# Autodesk Inventor assembly: martro_hettlich
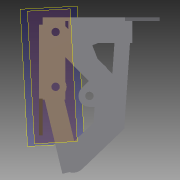
[picture p0: Inventor's stored thumbnail of the model, 180x180]
Saved by Autodesk Inventor 2015 SP1 (Build 190203100, 203)
## iProperties
Created: 2015-03-29
Part Number: martro_hettlich
Document SubType Name: Assembly
Designer: Marcin
Author: Marcin
## Documents named in this file (8)
- C:\Users\Marcin\Documents\Inventor\SynerGolf\zawias\martro_hettlich.iam
- C:\Users\Marcin\Documents\Inventor\SynerGolf\zawias\hettich_1.ipt
- C:\Users\Marcin\Documents\Inventor\SynerGolf\zawias\hettlich_2.ipt
- C:\Users\Marcin\Documents\Inventor\SynerGolf\zawias\hettlich_3.ipt
- C:\Users\Marcin\Documents\Inventor\SynerGolf\zawias\hettlich_4.ipt
- C:\Users\Marcin\Documents\Inventor\SynerGolf\zawias\hettlich_5.ipt
- C:\Users\Marcin\Documents\Inventor\SynerGolf\zawias\hettlich_6.ipt
- C:\Users\Marcin\Documents\Inventor\SynerGolf\parameters.xlsx
## Components (6 placed, 6 different names)
1. hettich_1:1 — Zestawiający:18, Zestawiający:20, Kąt:1, Zestawiający:22, Zestawiający:23, Zestawiający:24
2. hettlich_2:1 — Zestawiający:7, Zestawiający:8, Zestawiający:13, Zestawiający:18, Zestawiający:20, Zestawiający:21
3. hettlich_4:1 — Zestawiający:7, Zestawiający:8, Zestawiający:10, Zestawiający:11, Zestawiający:25
4. hettlich_5:1 — Zestawiający:10, Zestawiający:11, Zestawiający:14, Równoległy:3, Równoległy:4, Kąt:1
5. hettlich_6:1 — Zestawiający:13, Zestawiający:14, Zestawiający:21
6. hettlich_3:1 — Zestawiający:23, Zestawiający:24, Zestawiający:25
## Relationships (18: Mate 14, Flush 2, Symmetry 1, Angle 1)
- Zestawiający:7 [Mate]: hettlich_2:1 ↔ hettlich_4:1
- Zestawiający:8 [Mate] (0.4 mm): hettlich_2:1 ↔ hettlich_4:1
- Zestawiający:10 [Mate]: hettlich_4:1 ↔ hettlich_5:1
- Zestawiający:11 [Mate] (0.4 mm): hettlich_4:1 ↔ hettlich_5:1
- Zestawiający:13 [Mate]: hettlich_2:1 ↔ hettlich_6:1
- Zestawiający:14 [Mate]: hettlich_5:1 ↔ hettlich_6:1
- Równoległy:3 [Flush]: hettlich_5:1
- Równoległy:4 [Flush]: hettlich_5:1
- Symetria:1 [Symmetry]
- Zestawiający:17 [Mate]
- Zestawiający:18 [Mate]: hettich_1:1 ↔ hettlich_2:1
- Zestawiający:20 [Mate]: hettich_1:1 ↔ hettlich_2:1
- Zestawiający:21 [Mate]: hettlich_2:1 ↔ hettlich_6:1
- Kąt:1 [Angle] (45 deg): hettich_1:1 ↔ hettlich_5:1
- Zestawiający:22 [Mate]: hettich_1:1
- Zestawiający:23 [Mate]: hettich_1:1 ↔ hettlich_3:1
- Zestawiający:24 [Mate]: hettich_1:1 ↔ hettlich_3:1
- Zestawiający:25 [Mate]: hettlich_4:1 ↔ hettlich_3:1
## Named parameters: angle = 45 deg
